# Autodesk Inventor assembly: Sax Cart
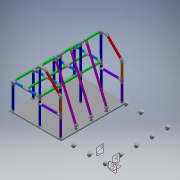
[picture p0: Inventor's stored thumbnail of the model, 180x180]
Saved by Autodesk Inventor 2018.2 (Build 222227000, 227)
## iProperties
Created: 2018-01-30
Part Number: Sax Cart
Document SubType Name: Assembly
Designer: owner
Author: owner
## Documents named in this file (23)
- Z:\The Pickle\Final Carts\Sax Cart\Sax Cart.iam
- Z:\The Pickle\Final Carts\Sax Cart\Plywood base - sax.ipt
- Z:\The Pickle\Inventor Pipe Parts\Formufit Fittings\Wood Mount 1 Inch.ipt
- Z:\The Pickle\Inventor Pipe Parts\Formufit Fittings\Tee 1 Inch.ipt
- Z:\The Pickle\Inventor Pipe Parts\Formufit Fittings\Slip Tee 1 Inch.ipt
- Z:\The Pickle\Inventor Pipe Parts\Formufit Fittings\45 Elbow 1 Inch.ipt
- Z:\The Pickle\Inventor Pipe Parts\Formufit Fittings\4-way Tee 1 Inch.ipt
- Z:\The Pickle\Inventor Pipe Parts\Formufit Fittings\Cross 1 Inch.ipt
- Z:\The Pickle\Inventor Pipe Parts\Formufit Fittings\5-way 1 Inch.ipt
- Z:\The Pickle\Final Carts\Sax Cart\Pipe 1.ipt
- Z:\The Pickle\Final Carts\Sax Cart\Pipe 2.ipt
- Z:\The Pickle\Final Carts\Sax Cart\Pipe 3.ipt
- Z:\The Pickle\Final Carts\Sax Cart\Pipe 4.ipt
- Z:\The Pickle\Final Carts\Sax Cart\Pipe 5.ipt
- Z:\The Pickle\Final Carts\Sax Cart\Pipe 6.ipt
- Z:\The Pickle\Final Carts\Sax Cart\Pipe 7.ipt
- Z:\The Pickle\Inventor Pipe Parts\Formufit Fittings\3-way 90 1 Inch.ipt
- Z:\The Pickle\Inventor Pipe Parts\Formufit Fittings\Formufit Pipe 1 Inch Flush Fittings.ipt
- Z:\The Pickle\Final Carts\Sax Cart\Pipe OD - ID adapt.ipt
- Z:\The Pickle\Final Carts\Sax Cart\Adjustable Elbow 1 Inch - Sax Angle.iam
- Z:\The Pickle\Inventor Pipe Parts\Lock Ideas\Eyebolt.ipt
- Z:\The Pickle\Inventor Pipe Parts\Lock Ideas\Eyebolt Nut.ipt
- Z:\The Pickle\Final Carts\Sax Cart\Sax Wheel.ipt
## Components (114 placed, 22 different names)
1. Plywood base - sax:1 — Mate:1, Tangent:2, Mate:2, Mate:3, Tangent:3, Flush:6
2. Wood Mount 1 Inch:1 — Mate:1, Tangent:2, Insert:1, Tangent:3
3. Wood Mount 1 Inch:2 — Insert:33
4. Wood Mount 1 Inch:3 — Insert:27, Mate:2
5. Wood Mount 1 Inch:4 — Insert:18
6. Wood Mount 1 Inch:5 — Insert:24
7. Wood Mount 1 Inch:6 — Insert:34
8. Wood Mount 1 Inch:7 — Insert:64
9. Wood Mount 1 Inch:8 — Insert:65
10. Wood Mount 1 Inch:9 — Insert:89
11. Wood Mount 1 Inch:10 — Insert:90
12. Wood Mount 1 Inch:11 — Insert:67
13. Wood Mount 1 Inch:12 — Insert:91
14. Wood Mount 1 Inch:13 — Insert:28, Mate:3
15. Tee 1 Inch:3 — Insert:20, Insert:21, Insert:55
16. Tee 1 Inch:4 — Insert:42, Insert:43
17. Tee 1 Inch:5 — Insert:74, Insert:75
18. Tee 1 Inch:6 — Insert:76, Insert:77
19. Tee 1 Inch:7 — Insert:16, Insert:17, Insert:86
20. Tee 1 Inch:8 — Insert:2, Insert:3, Insert:85
21. Slip Tee 1 Inch:1 — Insert:4, Flush:1
22. Slip Tee 1 Inch:2 — Flush:1, Insert:15
23. Slip Tee 1 Inch:3 — Insert:96, Insert:97, Angle:2, Angle:3, Insert:99
24. Slip Tee 1 Inch:4 — Insert:97, Angle:3, Insert:100
25. Slip Tee 1 Inch:5 — Angle:1, Insert:93, Insert:96, Insert:98
26. 45 Elbow 1 Inch:1 — Insert:87
27. 45 Elbow 1 Inch:2 — Insert:88
28. 4-way Tee 1 Inch:1 — Insert:12, Insert:30, Insert:71, Mate:7
29. 4-way Tee 1 Inch:2 — Insert:7, Insert:19, Insert:29, Insert:68, Mate:5
30. Cross 1 Inch:1 — Insert:45, Insert:46, Insert:57
31. Cross 1 Inch:2 — Insert:48, Insert:49, Insert:56
32. 5-way 1 Inch:1 — Insert:8, Insert:9, Insert:31, Insert:47, Insert:69
33. 5-way 1 Inch:2 — Insert:10, Insert:11, Insert:32, Insert:44, Insert:70
34. Pipe 1:1 — Insert:27, Insert:29
35. Pipe 1:2 — Insert:28, Insert:30
36. Pipe 1:3 — Insert:24, Insert:51, Cylindrical:2
37. Pipe 1:4 — Insert:31, Insert:33
38. Pipe 1:5 — Insert:32, Insert:34
39. Pipe 1:6 — Insert:62, Insert:64
40. Pipe 1:7 — Insert:63, Insert:65
41. Pipe 1:8 — Insert:66, Insert:67, Cylindrical:3
42. Pipe 1:9 — Insert:68, Insert:72, Angle:1, Angle:2, Cylindrical:1
43. Pipe 1:10 — Insert:69
44. Pipe 1:11 — Insert:70
45. Pipe 1:12 — Insert:71, Cylindrical:4
46. Pipe 2:1 — Insert:7, Insert:8
47. Pipe 2:2 — Insert:59, Insert:60
48. Pipe 2:3 — Insert:53, Insert:61
49. Pipe 2:4 — Insert:73, Insert:74
50. Pipe 2:5 — Insert:75, Insert:76
51. Pipe 2:6 — Insert:77, Insert:78
52. Pipe 2:7 — Insert:57
53. Pipe 2:8 — Insert:56
54. Pipe 2:9 — Insert:55
55. Pipe 2:10 — Insert:52, Insert:58
56. Pipe 2:11 — Insert:11, Insert:12
57. Pipe 2:12 — Insert:9, Insert:10
58. Pipe 3:1 — Insert:1, Insert:2
59. Pipe 3:2 — Insert:17, Insert:18
60. Pipe 3:3 — Insert:3, Insert:4
61. Pipe 3:4 — Insert:15, Insert:16
62. Pipe 4:1 — Insert:100, Insert:106
63. Pipe 4:2 — Insert:99, Insert:104
64. Pipe 4:3 — Insert:98, Insert:102
65. Pipe 5:1 — Insert:21, Insert:50
66. Pipe 5:2 — Insert:42, Insert:54
67. Pipe 5:3 — Insert:43
68. Pipe 5:4 — Insert:44, Insert:45
69. Pipe 5:5 — Insert:46
70. Pipe 5:6 — Insert:47, Insert:48
71. Pipe 5:7 — Insert:49
72. Pipe 5:8 — Insert:19, Insert:20
73. Pipe 6:1 — Insert:84
74. Pipe 6:2 — Insert:83
75. Pipe 7:1 — Insert:85, Insert:87
76. Pipe 7:2 — Insert:86, Insert:88
77. 3-way 90 1 Inch:1 — Insert:72, Insert:73, Insert:79, Insert:93, Mate:6
78. 3-way 90 1 Inch:2 — Insert:50, Insert:51, Insert:52, Mate:4
79. 3-way 90 1 Inch:3 — Insert:53, Insert:54, Insert:66, Mate:8
80. 3-way 90 1 Inch:4 — Insert:78, Insert:81, Mate:9
81. 4-way Tee 1 Inch:3 — Insert:58, Insert:59, Insert:62
82. 4-way Tee 1 Inch:4 — Insert:60, Insert:61, Insert:63
83. 45 Elbow 1 Inch:3 — Insert:82, Insert:84
84. 45 Elbow 1 Inch:4 — Insert:80, Insert:83
85. Formufit Pipe 1 Inch Flush Fittings:1 — Insert:79, Insert:80
86. Formufit Pipe 1 Inch Flush Fittings:2 — Insert:81, Insert:82
87. Pipe OD - ID adapt:2 — Insert:89, Insert:101
88. Pipe OD - ID adapt:3 — Insert:90, Insert:103
89. Pipe OD - ID adapt:4 — Insert:91, Insert:105
90. Adjustable Elbow 1 Inch - Sax Angle:2 [sub-assembly] — Insert:101, Insert:102
91. Adjustable Elbow 1 Inch - Sax Angle:3 [sub-assembly] — Insert:103, Insert:104
92. Adjustable Elbow 1 Inch - Sax Angle:4 [sub-assembly] — Insert:105, Insert:106
93. Eyebolt:1 — Cylindrical:1, Cylindrical:8
94. Eyebolt:2 — Cylindrical:2, Cylindrical:5
95. Eyebolt:3 — Cylindrical:3, Cylindrical:7
96. Eyebolt:4 — Cylindrical:4, Cylindrical:6
97. Eyebolt Nut:1 — Cylindrical:5
98. Eyebolt Nut:2 — Cylindrical:6
99. Eyebolt Nut:3 — Cylindrical:7
100. Eyebolt Nut:4 — Cylindrical:8
101. Sax Wheel:1 — Flush:5, Flush:10, Mate:13, Flush:20
102. Sax Wheel:2 — Flush:4, Flush:5, Flush:9, Flush:10, Mate:12, Mate:13, Flush:23
103. Sax Wheel:3 — Flush:3, Flush:4, Flush:8, Flush:9, Mate:11, Mate:12, Flush:24
104. Sax Wheel:4 — Flush:2, Flush:3, Flush:7, Flush:8, Mate:10, Mate:11, Flush:28
105. Sax Wheel:5 — Flush:2, Flush:6, Flush:7, Mate:10, Flush:11, Flush:31
106. Sax Wheel:6 — Flush:11, Flush:22, Flush:35, Mate:14
107. Sax Wheel:8 — Flush:14, Flush:25, Flush:29, Flush:30
108. Sax Wheel:9 — Flush:14, Flush:15, Flush:25, Flush:32
109. Sax Wheel:10 — Flush:15, Flush:16, Flush:28, Flush:32, Flush:33
110. Sax Wheel:11 — Flush:16, Flush:17, Flush:24, Flush:33, Flush:34
111. Sax Wheel:12 — Flush:17, Flush:18, Flush:23, Flush:34, Flush:35
112. Sax Wheel:13 — Flush:18, Flush:19, Flush:21, Flush:22, Mate:14, Mate:15
113. Sax Wheel:14 — Flush:19, Flush:20, Flush:21, Mate:15
114. Sax Wheel:15 — Flush:29, Flush:30, Flush:31
## Relationships (147: Insert 88, Flush 31, Mate 15, CylindricalJoint 8, Angle 3, Tangent 2)
- Mate:1: Plywood base - sax:1 ↔ Wood Mount 1 Inch:1
- Tangent:2: Plywood base - sax:1 ↔ Wood Mount 1 Inch:1
- Insert:1: Wood Mount 1 Inch:1 ↔ Pipe 3:1
- Insert:2: Tee 1 Inch:8 ↔ Pipe 3:1
- Insert:3: Tee 1 Inch:8 ↔ Pipe 3:3
- Insert:4: Slip Tee 1 Inch:1 ↔ Pipe 3:3
- Insert:7: 4-way Tee 1 Inch:2 ↔ Pipe 2:1
- Insert:8: 5-way 1 Inch:1 ↔ Pipe 2:1
- Insert:9: 5-way 1 Inch:1 ↔ Pipe 2:12
- Insert:10: 5-way 1 Inch:2 ↔ Pipe 2:12
- Insert:11: 5-way 1 Inch:2 ↔ Pipe 2:11
- Insert:12: 4-way Tee 1 Inch:1 ↔ Pipe 2:11
- Flush:1: Slip Tee 1 Inch:1 ↔ Slip Tee 1 Inch:2
- Insert:15: Slip Tee 1 Inch:2 ↔ Pipe 3:4
- Insert:16: Tee 1 Inch:7 ↔ Pipe 3:4
- Insert:17: Tee 1 Inch:7 ↔ Pipe 3:2
- Insert:18: Wood Mount 1 Inch:4 ↔ Pipe 3:2
- Insert:19: 4-way Tee 1 Inch:2 ↔ Pipe 5:8
- Insert:20: Tee 1 Inch:3 ↔ Pipe 5:8
- Insert:21: Tee 1 Inch:3 ↔ Pipe 5:1
- Insert:24: Wood Mount 1 Inch:5 ↔ Pipe 1:3
- Insert:27: Wood Mount 1 Inch:3 ↔ Pipe 1:1
- Mate:2: Plywood base - sax:1 ↔ Wood Mount 1 Inch:3
- Insert:28: Wood Mount 1 Inch:13 ↔ Pipe 1:2
- Mate:3: Plywood base - sax:1 ↔ Wood Mount 1 Inch:13
- Insert:29: 4-way Tee 1 Inch:2 ↔ Pipe 1:1
- Insert:30: 4-way Tee 1 Inch:1 ↔ Pipe 1:2
- Insert:31: 5-way 1 Inch:1 ↔ Pipe 1:4
- Insert:32: 5-way 1 Inch:2 ↔ Pipe 1:5
- Insert:33: Wood Mount 1 Inch:2 ↔ Pipe 1:4
- Insert:34: Wood Mount 1 Inch:6 ↔ Pipe 1:5
- Insert:42: Tee 1 Inch:4 ↔ Pipe 5:2
- Insert:43: Tee 1 Inch:4 ↔ Pipe 5:3
- Insert:44: 5-way 1 Inch:2 ↔ Pipe 5:4
- Insert:45: Cross 1 Inch:1 ↔ Pipe 5:4
- Insert:46: Cross 1 Inch:1 ↔ Pipe 5:5
- Insert:47: 5-way 1 Inch:1 ↔ Pipe 5:6
- Insert:48: Cross 1 Inch:2 ↔ Pipe 5:6
- Insert:49: Cross 1 Inch:2 ↔ Pipe 5:7
- Insert:50: Pipe 5:1 ↔ 3-way 90 1 Inch:2
- Insert:51: Pipe 1:3 ↔ 3-way 90 1 Inch:2
- Insert:52: Pipe 2:10 ↔ 3-way 90 1 Inch:2
- Insert:53: Pipe 2:3 ↔ 3-way 90 1 Inch:3
- Insert:54: Pipe 5:2 ↔ 3-way 90 1 Inch:3
- Insert:55: Tee 1 Inch:3 ↔ Pipe 2:9
- Insert:56: Cross 1 Inch:2 ↔ Pipe 2:8
- Insert:57: Cross 1 Inch:1 ↔ Pipe 2:7
- Insert:58: Pipe 2:10 ↔ 4-way Tee 1 Inch:3
- Insert:59: Pipe 2:2 ↔ 4-way Tee 1 Inch:3
- Insert:60: Pipe 2:2 ↔ 4-way Tee 1 Inch:4
- Insert:61: Pipe 2:3 ↔ 4-way Tee 1 Inch:4
- Insert:62: Pipe 1:6 ↔ 4-way Tee 1 Inch:3
- Insert:63: Pipe 1:7 ↔ 4-way Tee 1 Inch:4
- Insert:64: Wood Mount 1 Inch:7 ↔ Pipe 1:6
- Insert:65: Wood Mount 1 Inch:8 ↔ Pipe 1:7
- Insert:66: Pipe 1:8 ↔ 3-way 90 1 Inch:3
- Insert:67: Wood Mount 1 Inch:11 ↔ Pipe 1:8
- Insert:68: 4-way Tee 1 Inch:2 ↔ Pipe 1:9
- Insert:69: 5-way 1 Inch:1 ↔ Pipe 1:10
- Insert:70: 5-way 1 Inch:2 ↔ Pipe 1:11
- Insert:71: 4-way Tee 1 Inch:1 ↔ Pipe 1:12
- Insert:72: Pipe 1:9 ↔ 3-way 90 1 Inch:1
- Insert:73: Pipe 2:4 ↔ 3-way 90 1 Inch:1
- Insert:74: Tee 1 Inch:5 ↔ Pipe 2:4
- Insert:75: Tee 1 Inch:5 ↔ Pipe 2:5
- Insert:76: Tee 1 Inch:6 ↔ Pipe 2:5
- Insert:77: Tee 1 Inch:6 ↔ Pipe 2:6
- Insert:78: Pipe 2:6 ↔ 3-way 90 1 Inch:4
- Insert:79: 3-way 90 1 Inch:1 ↔ Formufit Pipe 1 Inch Flush Fittings:1
- Insert:80: 45 Elbow 1 Inch:4 ↔ Formufit Pipe 1 Inch Flush Fittings:1
- Insert:81: 3-way 90 1 Inch:4 ↔ Formufit Pipe 1 Inch Flush Fittings:2
- Insert:82: 45 Elbow 1 Inch:3 ↔ Formufit Pipe 1 Inch Flush Fittings:2
- Insert:83: Pipe 6:2 ↔ 45 Elbow 1 Inch:4
- Insert:84: Pipe 6:1 ↔ 45 Elbow 1 Inch:3
- Insert:85: Tee 1 Inch:8 ↔ Pipe 7:1
- Insert:86: Tee 1 Inch:7 ↔ Pipe 7:2
- Insert:87: 45 Elbow 1 Inch:1 ↔ Pipe 7:1
- Insert:88: 45 Elbow 1 Inch:2 ↔ Pipe 7:2
- Insert:89: Wood Mount 1 Inch:9 ↔ Pipe OD - ID adapt:2
- Insert:90: Wood Mount 1 Inch:10 ↔ Pipe OD - ID adapt:3
- Insert:91: Wood Mount 1 Inch:12 ↔ Pipe OD - ID adapt:4
- Angle:1 (23.14 deg): Slip Tee 1 Inch:5 ↔ Pipe 1:9
- Insert:93 (204.7875 mm): Slip Tee 1 Inch:5 ↔ 3-way 90 1 Inch:1
- Insert:96 (234.95 mm): Slip Tee 1 Inch:3 ↔ Slip Tee 1 Inch:5
- Insert:97 (234.95 mm): Slip Tee 1 Inch:3 ↔ Slip Tee 1 Inch:4
- Angle:2 (23.14 deg): Slip Tee 1 Inch:3 ↔ Pipe 1:9
- Angle:3 (0 deg): Slip Tee 1 Inch:3 ↔ Slip Tee 1 Inch:4
- Insert:98: Slip Tee 1 Inch:5 ↔ Pipe 4:3
- Insert:99: Slip Tee 1 Inch:3 ↔ Pipe 4:2
- Insert:100: Slip Tee 1 Inch:4 ↔ Pipe 4:1
- Insert:101: Pipe OD - ID adapt:2 ↔ Adjustable Elbow 1 Inch - Sax Angle:2
- Insert:102: Pipe 4:3 ↔ Adjustable Elbow 1 Inch - Sax Angle:2
- Insert:103: Pipe OD - ID adapt:3 ↔ Adjustable Elbow 1 Inch - Sax Angle:3
- Insert:104: Pipe 4:2 ↔ Adjustable Elbow 1 Inch - Sax Angle:3
- Insert:105: Pipe OD - ID adapt:4 ↔ Adjustable Elbow 1 Inch - Sax Angle:4
- Insert:106: Pipe 4:1 ↔ Adjustable Elbow 1 Inch - Sax Angle:4
- Mate:4: 3-way 90 1 Inch:2
- Mate:5: 4-way Tee 1 Inch:2
- Mate:6: 3-way 90 1 Inch:1
- Mate:7: 4-way Tee 1 Inch:1
- Mate:8: 3-way 90 1 Inch:3
- Mate:9: 3-way 90 1 Inch:4
- Cylindrical:1: Pipe 1:9 ↔ Eyebolt:1
- Cylindrical:2: Pipe 1:3 ↔ Eyebolt:2
- Cylindrical:3: Pipe 1:8 ↔ Eyebolt:3
- Cylindrical:4: Pipe 1:12 ↔ Eyebolt:4
- Cylindrical:5: Eyebolt:2 ↔ Eyebolt Nut:1
- Cylindrical:6: Eyebolt:4 ↔ Eyebolt Nut:2
- Cylindrical:7: Eyebolt:3 ↔ Eyebolt Nut:3
- Cylindrical:8: Eyebolt:1 ↔ Eyebolt Nut:4
- Tangent:3: Plywood base - sax:1 ↔ Wood Mount 1 Inch:1
- Flush:2: Sax Wheel:4 ↔ Sax Wheel:5
- Flush:3: Sax Wheel:3 ↔ Sax Wheel:4
- Flush:4: Sax Wheel:2 ↔ Sax Wheel:3
- Flush:5: Sax Wheel:1 ↔ Sax Wheel:2
- Flush:6: Plywood base - sax:1 ↔ Sax Wheel:5
- Flush:7: Sax Wheel:4 ↔ Sax Wheel:5
- Flush:8: Sax Wheel:3 ↔ Sax Wheel:4
- Flush:9: Sax Wheel:2 ↔ Sax Wheel:3
- Flush:10: Sax Wheel:1 ↔ Sax Wheel:2
- Mate:10 (236.3026 mm): Sax Wheel:4 ↔ Sax Wheel:5
- Mate:11 (236.3026 mm): Sax Wheel:3 ↔ Sax Wheel:4
- Mate:12 (236.3026 mm): Sax Wheel:2 ↔ Sax Wheel:3
- Mate:13 (236.3026 mm): Sax Wheel:1 ↔ Sax Wheel:2
- Flush:11: Sax Wheel:5 ↔ Sax Wheel:6
- Flush:14: Sax Wheel:8 ↔ Sax Wheel:9
- Flush:15: Sax Wheel:9 ↔ Sax Wheel:10
- Flush:16: Sax Wheel:10 ↔ Sax Wheel:11
- Flush:17: Sax Wheel:11 ↔ Sax Wheel:12
- Flush:18: Sax Wheel:12 ↔ Sax Wheel:13
- Flush:19: Sax Wheel:13 ↔ Sax Wheel:14
- Flush:20: Sax Wheel:1 ↔ Sax Wheel:14
- Flush:21: Sax Wheel:13 ↔ Sax Wheel:14
- Flush:22: Sax Wheel:6 ↔ Sax Wheel:13
- Flush:23: Sax Wheel:2 ↔ Sax Wheel:12
- Flush:24: Sax Wheel:3 ↔ Sax Wheel:11
- Flush:25: Sax Wheel:8 ↔ Sax Wheel:9
- Flush:28: Sax Wheel:4 ↔ Sax Wheel:10
- Flush:29: Sax Wheel:8 ↔ Sax Wheel:15
- Flush:30: Sax Wheel:8 ↔ Sax Wheel:15
- Flush:31: Sax Wheel:5 ↔ Sax Wheel:15
- Flush:32: Sax Wheel:9 ↔ Sax Wheel:10
- Flush:33: Sax Wheel:10 ↔ Sax Wheel:11
- Flush:34: Sax Wheel:11 ↔ Sax Wheel:12
- Flush:35: Sax Wheel:6 ↔ Sax Wheel:12
- Mate:14 (207.5349 mm): Sax Wheel:6 ↔ Sax Wheel:13
- Mate:15 (207.5349 mm): Sax Wheel:13 ↔ Sax Wheel:14
